# Autodesk Inventor assembly: PhoneFlipper1-SFK
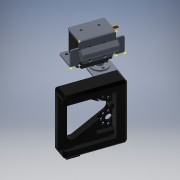
[picture p0: Inventor's stored thumbnail of the model, 180x180]
Saved by Autodesk Inventor 2017 (Build 210142000, 142)
## iProperties
Created: 2017-09-01
Part Number: PhoneFlipper1-SFK
Document SubType Name: Assembly
Designer: sfreisem-kirov
Author: sfreisem-kirov
## Documents named in this file (5)
- C:\Users\sfreisem-kirov\Documents\GitHub\ftc_app\Parts\phoneHolder\PhoneFlipper1-SFK.iam
- C:\Users\sfreisem-kirov\Documents\GitHub\ftc_app\Parts\phoneHolder\roundedLbracket1-SFK.ipt
- C:\Users\sfreisem-kirov\Documents\GitHub\ftc_app\Parts\phoneHolder\PhoneCase-SFK.ipt
- C:\Users\sfreisem-kirov\Documents\GitHub\ftc_app\Parts\phoneHolder\Servo.iam
- C:\Users\sfreisem-kirov\Desktop\servoHolder1-FK.ipt
## Components (4 placed, 4 different names)
1. PhoneCase-SFK:1 — Mate:1, Mate:2, Mate:3
2. roundedLbracket1-SFK:1 — Mate:1, Mate:2, Mate:3, Mate:4, Mate:5, Mate:6
3. Servo:1 [sub-assembly] — Mate:4, Mate:5, Mate:6, Mate:7, Mate:8, Mate:9
4. servoHolder1-FK:1 — Mate:7, Mate:8, Mate:9
## Relationships (9: Mate 9)
- Mate:1: PhoneCase-SFK:1 ↔ roundedLbracket1-SFK:1
- Mate:2: PhoneCase-SFK:1 ↔ roundedLbracket1-SFK:1
- Mate:3: PhoneCase-SFK:1 ↔ roundedLbracket1-SFK:1
- Mate:4: roundedLbracket1-SFK:1 ↔ Servo:1
- Mate:5: roundedLbracket1-SFK:1 ↔ Servo:1
- Mate:6: roundedLbracket1-SFK:1 ↔ Servo:1
- Mate:7: Servo:1 ↔ servoHolder1-FK:1
- Mate:8: Servo:1 ↔ servoHolder1-FK:1
- Mate:9: Servo:1 ↔ servoHolder1-FK:1
